# Autodesk Inventor assembly: The Claw
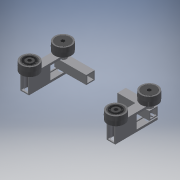
[picture p0: Inventor's stored thumbnail of the model, 180x180]
Saved by Autodesk Inventor 2018 (Build 220112000, 112)
## iProperties
Created: 2018-01-13
Part Number: The Claw
Document SubType Name: Assembly
Designer: Orangeracer
Author: Orangeracer
## iProperties of the stored document am-3436+2IN+Stealth,+375+Hex+Bore.ipt
Created: 2016-09-09
Part Number: am-3436+2IN+Stealth,+375+Hex+Bore
Material: Generic
Description: STEP AP214
Document SubType Name: Modeling
Designer: Orangeracer
Density: 1 g/cm^3
Appearance: Default
Sending System: SolidWorks 2014
Preprocessor: SwSTEP 2.0
Title: am-3436 2IN Stealth, 375 Hex Bore.STEP
Revision Number: ANY
## Documents named in this file (6)
- **E:\robot17'\2018 CAD Parts\CUBErt\The Claw.iam*LocalDocs*xBv1qztrgKexcehgyOgqxuglqKa*am-3436+2IN+Stealth,+375+Hex+Bore.ipt
- G:\robot17'\2018 CAD Parts\CUBErt\The Claw.iam
- G:\robot17'\2018 CAD Parts\CUBErt\C Arm.ipt
- **G:\robot17'\2018 CAD Parts\CUBErt\The Claw.iam*LocalDocs*xBv1qztrgKexcehgyOgqxuglqKa*am-3436+2IN+Stealth,+375+Hex+Bore.ipt
- G:\robot17'\2018 CAD Parts\CUBErt\C Spring load.ipt
- G:\robot17'\am-3436+2IN+Stealth,+375+Hex+Bore.STEP
## Components (8 placed, 3 different names)
1. C Arm:1 — Mate:22, Mate:23, Mate:28, Mate:29, Mate:35, Mate:36, Flush:18, Mate:37
2. C Arm:2 — Mate:16, Mate:17, Mate:30, Mate:31, Mate:32, Mate:33, Mate:34, Flush:19, Mate:37
3. am-3436+2IN+Stealth,+375+Hex+Bore:3 — Mate:22, Mate:23
4. am-3436+2IN+Stealth,+375+Hex+Bore:6 — Mate:16, Mate:17
5. am-3436+2IN+Stealth,+375+Hex+Bore:8 — Mate:30, Mate:31, Mate:32
6. am-3436+2IN+Stealth,+375+Hex+Bore:9 — Mate:28, Mate:29
7. C Spring load:1 — Mate:33, Mate:34, Flush:19, Flush:20, Flush:21
8. C Spring load:2 — Mate:35, Mate:36, Flush:18, Flush:20, Flush:21
## Relationships (18: Mate 14, Flush 4)
- Mate:16: C Arm:2 ↔ am-3436+2IN+Stealth,+375+Hex+Bore:6
- Mate:17: C Arm:2 ↔ am-3436+2IN+Stealth,+375+Hex+Bore:6
- Mate:22: C Arm:1 ↔ am-3436+2IN+Stealth,+375+Hex+Bore:3
- Mate:23: C Arm:1 ↔ am-3436+2IN+Stealth,+375+Hex+Bore:3
- Mate:28: C Arm:1 ↔ am-3436+2IN+Stealth,+375+Hex+Bore:9
- Mate:29: C Arm:1 ↔ am-3436+2IN+Stealth,+375+Hex+Bore:9
- Mate:30: C Arm:2 ↔ am-3436+2IN+Stealth,+375+Hex+Bore:8
- Mate:31: C Arm:2 ↔ am-3436+2IN+Stealth,+375+Hex+Bore:8
- Mate:32: C Arm:2 ↔ am-3436+2IN+Stealth,+375+Hex+Bore:8
- Mate:33: C Arm:2 ↔ C Spring load:1
- Mate:34 (6.35 mm): C Arm:2 ↔ C Spring load:1
- Mate:35: C Arm:1 ↔ C Spring load:2
- Mate:36 (6.35 mm): C Arm:1 ↔ C Spring load:2
- Flush:18: C Arm:1 ↔ C Spring load:2
- Flush:19: C Arm:2 ↔ C Spring load:1
- Flush:20: C Spring load:1 ↔ C Spring load:2
- Flush:21: C Spring load:1 ↔ C Spring load:2
- Mate:37 (228.6 mm): C Arm:1 ↔ C Arm:2
